# Autodesk Inventor assembly: Lap rap truc Y
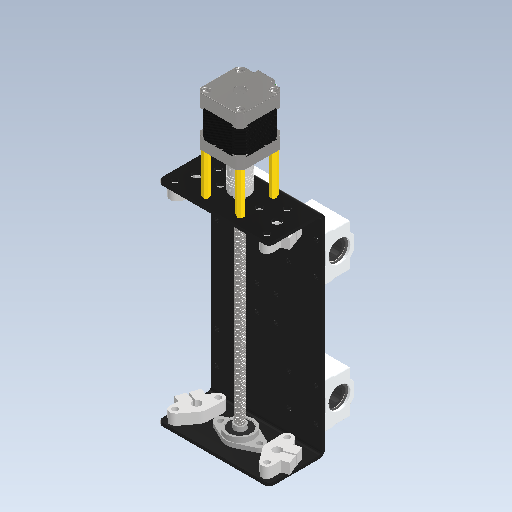
[picture p0: Inventor's stored thumbnail of the model, 512x512]
Saved by Autodesk Inventor 2020 (Build 240168000, 168)
## iProperties
Created: 2021-05-26
Part Number: Lap rap truc Y
Document SubType Name: Assembly
Designer: admin
Author: admin
## Documents named in this file (11)
- C:\Users\Admin\Downloads\CNC phay mach\Lap rap truc Y.iam
- C:\Users\Admin\Downloads\CNC phay mach\De  truc Y.ipt
- C:\Users\Admin\Downloads\CNC phay mach\Kep Truc KLF-08.ipt
- C:\Users\Admin\Downloads\CNC phay mach\Dong co Buoc\NEMA 17.iam
- C:\Users\Admin\Downloads\CNC phay mach\Tru dong 40mm.ipt
- C:\Users\Admin\Downloads\CNC phay mach\AoVitmeT8.ipt
- C:\Users\Admin\Downloads\CNC phay mach\SC12uu\PILLOW 12MM FINAL.iam
- C:\Users\Admin\Downloads\CNC phay mach\pcb-cnc-2.snapshot.25\T8 Nut.ipt
- C:\Users\Admin\Downloads\CNC phay mach\Flexible Coupling 8,8.ipt
- C:\Users\Admin\Downloads\CNC phay mach\Vitme T8 dai 200mm.ipt
- C:\Users\Admin\Downloads\CNC phay mach\SHF08.ipt
## Components (20 placed, 10 different names)
1. De  truc Y:1 — Mate:4, Mate:5, Mate:6, Mate:13, Mate:15, Mate:16, Mate:21, Mate:22, Mate:23, Mate:24, Mate:25, Mate:26, Mate:27, Mate:28, Mate:34, Mate:35, Mate:36, Mate:37, Mate:38, Mate:39, Mate:46, Mate:47, Mate:48, Mate:49, Mate:50, Mate:51, Mate:52, Mate:53, Mate:54, Mate:55, Mate:56, Mate:57, Mate:58, Mate:59, Mate:60, Mate:61, Mate:62, Mate:63, Mate:64, Mate:65
2. NEMA 17:1 [sub-assembly] — Mate:29, Mate:30, Mate:42, Mate:43, Mate:44
3. Kep Truc KLF-08:2 — Mate:4, Mate:5, Mate:6
4. Kep Truc KLF-08:3 — Mate:13, Mate:15, Mate:16, Mate:19
5. Vitme T8 dai 200mm:1 — Mate:19, Mate:45
6. Tru dong 40mm:1 — Mate:22, Mate:26, Mate:44
7. Tru dong 40mm:2 — Mate:21, Mate:25
8. Tru dong 40mm:3 — Mate:24, Mate:28, Mate:29
9. Tru dong 40mm:4 — Mate:23, Mate:27, Mate:30
10. AoVitmeT8:1 — Mate:34, Mate:35, Mate:36, Mate:40, Mate:41
11. PILLOW 12MM FINAL:5 [sub-assembly] — Mate:37, Mate:38, Mate:39
12. T8 Nut:1 — Mate:40, Mate:41
13. Flexible Coupling 8,8:1 — Mate:42, Mate:43, Mate:45
14. PILLOW 12MM FINAL:6 [sub-assembly] — Mate:46, Mate:47, Mate:48
15. PILLOW 12MM FINAL:7 [sub-assembly] — Flush:1, Flush:2, Mate:51, Mate:52, Mate:53
16. PILLOW 12MM FINAL:8 [sub-assembly] — Flush:1, Flush:2, Mate:49, Mate:50
17. SHF08:1 — Mate:54, Mate:55, Mate:56
18. SHF08:2 — Mate:60, Mate:61, Mate:62
19. SHF08:3 — Mate:63, Mate:64, Mate:65
20. SHF08:4 — Mate:57, Mate:58, Mate:59
## Relationships (51: Mate 49, Flush 2)
- Mate:4: De  truc Y:1 ↔ Kep Truc KLF-08:2
- Mate:5: De  truc Y:1 ↔ Kep Truc KLF-08:2
- Mate:6: De  truc Y:1 ↔ Kep Truc KLF-08:2
- Mate:13: De  truc Y:1 ↔ Kep Truc KLF-08:3
- Mate:15: De  truc Y:1 ↔ Kep Truc KLF-08:3
- Mate:16: De  truc Y:1 ↔ Kep Truc KLF-08:3
- Mate:19: Kep Truc KLF-08:3 ↔ Vitme T8 dai 200mm:1
- Mate:21: De  truc Y:1 ↔ Tru dong 40mm:2
- Mate:22: De  truc Y:1 ↔ Tru dong 40mm:1
- Mate:23: De  truc Y:1 ↔ Tru dong 40mm:4
- Mate:24: De  truc Y:1 ↔ Tru dong 40mm:3
- Mate:25: De  truc Y:1 ↔ Tru dong 40mm:2
- Mate:26: De  truc Y:1 ↔ Tru dong 40mm:1
- Mate:27: De  truc Y:1 ↔ Tru dong 40mm:4
- Mate:28: De  truc Y:1 ↔ Tru dong 40mm:3
- Mate:29: NEMA 17:1 ↔ Tru dong 40mm:3
- Mate:30: NEMA 17:1 ↔ Tru dong 40mm:4
- Mate:34: De  truc Y:1 ↔ AoVitmeT8:1
- Mate:35: De  truc Y:1 ↔ AoVitmeT8:1
- Mate:36: De  truc Y:1 ↔ AoVitmeT8:1
- Mate:37: De  truc Y:1 ↔ PILLOW 12MM FINAL:5
- Mate:38: De  truc Y:1 ↔ PILLOW 12MM FINAL:5
- Mate:39: De  truc Y:1 ↔ PILLOW 12MM FINAL:5
- Mate:40: AoVitmeT8:1 ↔ T8 Nut:1
- Mate:41: AoVitmeT8:1 ↔ T8 Nut:1
- Mate:42: NEMA 17:1 ↔ Flexible Coupling 8,8:1
- Mate:43 (-10 mm): NEMA 17:1 ↔ Flexible Coupling 8,8:1
- Mate:44: NEMA 17:1 ↔ Tru dong 40mm:1
- Mate:45 (-10 mm): Vitme T8 dai 200mm:1 ↔ Flexible Coupling 8,8:1
- Mate:46: De  truc Y:1 ↔ PILLOW 12MM FINAL:6
- Mate:47: De  truc Y:1 ↔ PILLOW 12MM FINAL:6
- Mate:48: De  truc Y:1 ↔ PILLOW 12MM FINAL:6
- Flush:1: PILLOW 12MM FINAL:7 ↔ PILLOW 12MM FINAL:8
- Flush:2: PILLOW 12MM FINAL:7 ↔ PILLOW 12MM FINAL:8
- Mate:49: De  truc Y:1 ↔ PILLOW 12MM FINAL:8
- Mate:50: De  truc Y:1 ↔ PILLOW 12MM FINAL:8
- Mate:51: De  truc Y:1 ↔ PILLOW 12MM FINAL:7
- Mate:52: De  truc Y:1 ↔ PILLOW 12MM FINAL:7
- Mate:53: De  truc Y:1 ↔ PILLOW 12MM FINAL:7
- Mate:54: De  truc Y:1 ↔ SHF08:1
- Mate:55: De  truc Y:1 ↔ SHF08:1
- Mate:56: De  truc Y:1 ↔ SHF08:1
- Mate:57: De  truc Y:1 ↔ SHF08:4
- Mate:58: De  truc Y:1 ↔ SHF08:4
- Mate:59: De  truc Y:1 ↔ SHF08:4
- Mate:60: De  truc Y:1 ↔ SHF08:2
- Mate:61: De  truc Y:1 ↔ SHF08:2
- Mate:62: De  truc Y:1 ↔ SHF08:2
- Mate:63: De  truc Y:1 ↔ SHF08:3
- Mate:64: De  truc Y:1 ↔ SHF08:3
- Mate:65: De  truc Y:1 ↔ SHF08:3
